# Autodesk Inventor assembly: Клапан2
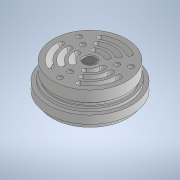
[picture p0: Inventor's stored thumbnail of the model, 180x180]
Saved by Autodesk Inventor 2021 (Build 250183000, 183)
## iProperties
Created: 2020-11-09
Part Number: Клапан2
Document SubType Name: Assembly
Designer: Тимоха
Author: Тимоха
## Documents named in this file (6)
- C:\Users\Тимоха\Desktop\КР Компрессор\МОЕ\Клапан2.iam
- C:\Users\Тимоха\Desktop\КР Компрессор\МОЕ\Мое седло.ipt
- C:\Users\Тимоха\Desktop\КР Компрессор\МОЕ\Мой ограничитель.ipt
- C:\Users\Тимоха\Desktop\КР Компрессор\МОЕ\Моя пластина.ipt
- C:\Users\Тимоха\Desktop\КР Компрессор\МОЕ\Клапан\Шпилька М24-6gx48 ГОСТ 22038-76.ipt
- C:\Users\Тимоха\Desktop\КР Компрессор\МОЕ\Клапан\Гайка М24-6H ГОСТ 5915-70.ipt
## Components (5 placed, 5 different names)
1. Мое седло:1 — С поворотом:1, С поворотом:2, С поворотом:4
2. Мой ограничитель:1 — С поворотом:1, С поворотом:3
3. Моя пластина:1 — С поворотом:2
4. Шпилька М24-6gx48 ГОСТ 22038-76:1 — С поворотом:3
5. Гайка М24-6H ГОСТ 5915-70:1 — С поворотом:4
## Relationships (4: RevoluteJoint 4)
- С поворотом:1 [RevoluteJoint]: Мое седло:1 ↔ Мой ограничитель:1
- С поворотом:2 [RevoluteJoint]: Мое седло:1 ↔ Моя пластина:1
- С поворотом:3 [RevoluteJoint]: Мой ограничитель:1 ↔ Шпилька М24-6gx48 ГОСТ 22038-76:1
- С поворотом:4 [RevoluteJoint]: Мое седло:1 ↔ Гайка М24-6H ГОСТ 5915-70:1
